# Autodesk Inventor assembly: Cup_Dispenser_Dynamic
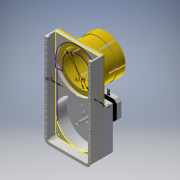
[picture p0: Inventor's stored thumbnail of the model, 180x180]
Saved by Autodesk Inventor 2016 (Build 200138000, 138)
## iProperties
Created: 2015-07-09
Part Number: Cup_Dispenser_Dynamic
Document SubType Name: Assembly
Designer: marku
Author: marku
## Documents named in this file (6)
- C:\Users\marku\Documents\GitHub\BarBot\Conception\Mechanical\Cup_Dispenser_Dynamic\Cup_Dispenser_Dynamic.iam
- C:\Users\marku\Documents\GitHub\BarBot\Conception\Mechanical\Cup_Dispenser_Dynamic\Cup_Dispenser_Hull.ipt
- C:\Users\marku\Documents\GitHub\BarBot\Conception\Mechanical\Cup_Dispenser_Dynamic\Cup_Dispenser_Fixture.ipt
- C:\Users\marku\Documents\GitHub\BarBot\Conception\Mechanical\Cup_Dispenser_Dynamic\Cup_Dispenser_Stepper_Montage.ipt
- C:\Users\marku\Documents\GitHub\BarBot\Conception\Mechanical\Cup_Dispenser_Dynamic\M1173041- NEMA 17.ipt
- C:\Users\marku\Documents\GitHub\BarBot\Conception\Mechanical\Cup_Dispenser_Dynamic\Cup_Dispenser_Slider.ipt
## Components (5 placed, 5 different names)
1. Cup_Dispenser_Hull:1 — Flush:1, Flush:2, Flush:3
2. Cup_Dispenser_Fixture:1 — Flush:1
3. Cup_Dispenser_Stepper_Montage:1 — Flush:2, Rigid:1
4. M1173041- NEMA 17:1 — Rigid:1
5. Cup_Dispenser_Slider:1 — Flush:3
## Relationships (4: Flush 3, WeldJoint 1)
- Flush:1: Cup_Dispenser_Hull:1 ↔ Cup_Dispenser_Fixture:1
- Flush:2: Cup_Dispenser_Hull:1 ↔ Cup_Dispenser_Stepper_Montage:1
- Rigid:1 [WeldJoint]: Cup_Dispenser_Stepper_Montage:1 ↔ M1173041- NEMA 17:1
- Flush:3: Cup_Dispenser_Hull:1 ↔ Cup_Dispenser_Slider:1
